# Autodesk Inventor assembly: Ensamble_4
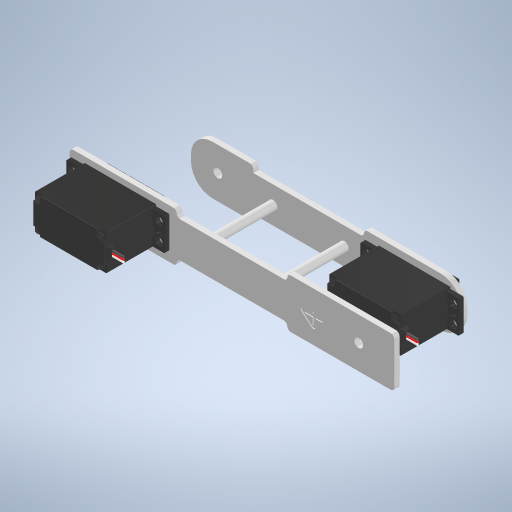
[picture p0: Inventor's stored thumbnail of the model, 512x512]
Saved by Autodesk Inventor 2023 (Build 270158000, 158)
## iProperties
Created: 2024-09-27
Part Number: Ensamble_4
Document SubType Name: Assembly
Designer: sebas
Author: sebas
## Documents named in this file (3)
- C:\Users\sebas\OneDrive\Documentos\ILLERO_MODELADO_ROBOT\Ensamble_4.iam
- C:\Users\sebas\OneDrive\Documentos\ILLERO_MODELADO_ROBOT\Pieza_eslabon_4.ipt
- C:\Users\sebas\OneDrive\Documentos\ILLERO_MODELADO_ROBOT\User Library-Subasa Servo S3003.ipt
## Components (3 placed, 2 different names)
1. Pieza_eslabon_4:1 — Coincidencia:25, Coincidencia:26, Coincidencia:27, Coincidencia:29, Coincidencia:30, Coincidencia:31, Coincidencia:32, Coincidencia:33
2. User Library-Subasa Servo S3003:3 — Coincidencia:25, Coincidencia:26, Coincidencia:27
3. User Library-Subasa Servo S3003:6 — Coincidencia:29, Coincidencia:30, Coincidencia:31
## Relationships (8: Mate 8)
- Coincidencia:25 [Mate]: Pieza_eslabon_4:1 ↔ User Library-Subasa Servo S3003:3
- Coincidencia:26 [Mate]: Pieza_eslabon_4:1 ↔ User Library-Subasa Servo S3003:3
- Coincidencia:27 [Mate]: Pieza_eslabon_4:1 ↔ User Library-Subasa Servo S3003:3
- Coincidencia:29 [Mate]: Pieza_eslabon_4:1 ↔ User Library-Subasa Servo S3003:6
- Coincidencia:30 [Mate]: Pieza_eslabon_4:1 ↔ User Library-Subasa Servo S3003:6
- Coincidencia:31 [Mate]: Pieza_eslabon_4:1 ↔ User Library-Subasa Servo S3003:6
- Coincidencia:32 [Mate]: Pieza_eslabon_4:1
- Coincidencia:33 [Mate]: Pieza_eslabon_4:1
